# Autodesk Inventor assembly: Dribler-Desmontable
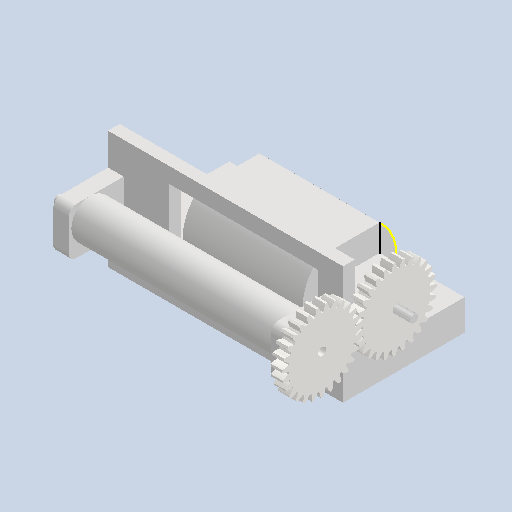
[picture p0: Inventor's stored thumbnail of the model, 512x512]
Saved by Autodesk Inventor 2024.2 (Build 282272000, 272)
## iProperties
Created: 2023-12-01
Part Number: Dribler-Desmontable
Document SubType Name: Assembly
Designer: felip
Author: felip
## Documents named in this file (6)
- C:\Users\felip\Documentos\Robocupp-Mecanica\Gemelo Digital V2\Dribler-Desmontable.iam
- C:\Users\felip\Documentos\Robocupp-Mecanica\Gemelo Digital V2\Base-Configurable-Dribler.ipt
- C:\Users\felip\Documentos\Robocupp-Mecanica\Gemelo Digital V2\Dc-Motor.ipt
- C:\Users\felip\Documentos\Robocupp-Mecanica\Gemelo Digital V2\Engranajes-Dribler\Design Accelerator\Engranaje A.ipt
- C:\Users\felip\Documentos\Robocupp-Mecanica\Gemelo Digital V2\Engranajes-Dribler\Design Accelerator\Engranaje B.ipt
- C:\Users\felip\Documentos\Robocupp-Mecanica\Gemelo Digital V2\Engranajes-Dribler\Design Accelerator\PseudoRoller.ipt
## Components (5 placed, 5 different names)
1. Base-Configurable-Dribler:1 — Rotational:1, Rotational:2, Rotational:3, Rotational:4
2. Dc-Motor:1 — Rotational:1
3. Spur Gear1:1 — Rotational:4
4. Spur Gear2:1 — Rotational:3
5. PseudoRoller:1 — Rotational:2
## Relationships (4: RevoluteJoint 4)
- Rotational:1 [RevoluteJoint]: Base-Configurable-Dribler:1 ↔ Dc-Motor:1
- Rotational:2 [RevoluteJoint]: Base-Configurable-Dribler:1 ↔ PseudoRoller:1
- Rotational:3 [RevoluteJoint]: Base-Configurable-Dribler:1 ↔ Spur Gear2:1
- Rotational:4 [RevoluteJoint]: Base-Configurable-Dribler:1 ↔ Spur Gear1:1
